# Autodesk Inventor assembly: 前腕_1
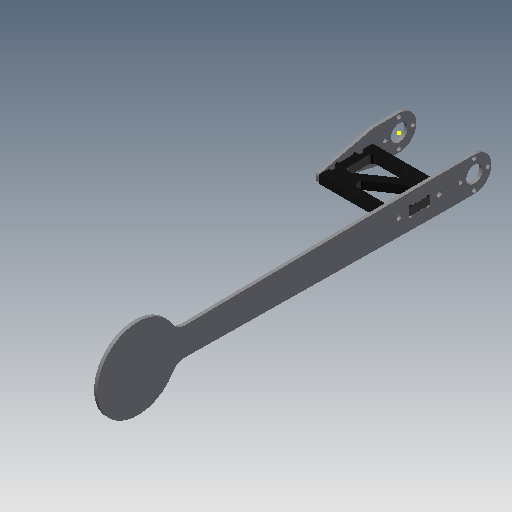
[picture p0: Inventor's stored thumbnail of the model, 512x512]
Saved by Autodesk Inventor 2017.3 (Build 213256000, 256)
## iProperties
Created: 2016-05-04
Part Number: 前腕_1
Document SubType Name: Assembly
Designer: hiroaki
Mass: 26.6275 g
Surface Area: 157.739 cm^2
Volume: 17.3877 cm^3
Density: 1.5314 g/cm^3
Author: hiroaki
## Documents named in this file (4)
- C:\Users\haya\Desktop\差分\171119OpenPlatform_設計\OpenPlatform ver.1.0\上半身\腕\前腕_1.iam
- C:\Users\haya\Desktop\差分\171119OpenPlatform_設計\OpenPlatform ver.1.0\上半身\腕\前腕_メインフレーム_1_1.ipt
- C:\Users\haya\Desktop\差分\171119OpenPlatform_設計\OpenPlatform ver.1.0\上半身\腕\前腕_サブフレーム_1_1.ipt
- C:\Users\haya\Desktop\差分\171119OpenPlatform_設計\OpenPlatform ver.1.0\上半身\腕\前腕_メインフレーム_1_2.ipt
## Components (3 placed, 3 different names)
1. 前腕_メインフレーム_1_1:1 — 挿入:3, 挿入:4
2. 前腕_サブフレーム_1_1:1 — メイト:1, メイト:2, フラッシュ:1, 挿入:3, 挿入:4, 挿入:5, 挿入:6
3. 前腕_メインフレーム_1_2:1 — 挿入:5, 挿入:6
## Relationships (7: Insert 4, Mate 2, Flush 1)
- メイト:1 [Mate]: 前腕_サブフレーム_1_1:1
- メイト:2 [Mate]: 前腕_サブフレーム_1_1:1
- フラッシュ:1 [Flush]: 前腕_サブフレーム_1_1:1
- 挿入:3 [Insert]: 前腕_メインフレーム_1_1:1 ↔ 前腕_サブフレーム_1_1:1
- 挿入:4 [Insert]: 前腕_メインフレーム_1_1:1 ↔ 前腕_サブフレーム_1_1:1
- 挿入:5 [Insert]: 前腕_サブフレーム_1_1:1 ↔ 前腕_メインフレーム_1_2:1
- 挿入:6 [Insert]: 前腕_サブフレーム_1_1:1 ↔ 前腕_メインフレーム_1_2:1
